# Autodesk Inventor assembly: underbrink_lite_asm_2
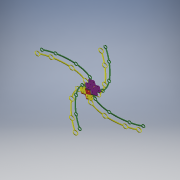
[picture p0: Inventor's stored thumbnail of the model, 180x180]
Saved by Autodesk Inventor 2019 (Build 230136000, 136)
## iProperties
Created: 2019-07-10
Part Number: underbrink_lite_asm_2
Document SubType Name: Assembly
Designer: Lino P
Mass: 5720.64 g
Surface Area: 2268.18 cm^2
Volume: 727.519 cm^3
Density: 7.86322 g/cm^3
Author: Lino P
## Documents named in this file (5)
- C:\Users\Lino P\Documents\000 - USFQ\TesisDev\ipt\underbrink_lite_asm_2.iam
- C:\Users\Lino P\Documents\000 - USFQ\TesisDev\ipt\underbrink_arm_lite_2.ipt
- C:\Users\Lino P\Documents\000 - USFQ\TesisDev\ipt\underbrink_base_lite.ipt
- C:\Users\Lino P\Documents\000 - USFQ\TesisDev\ipt\underbrink_arm_lite_2_bigDiam.ipt
- C:\Users\Lino P\Documents\000 - USFQ\TesisDev\ipt\underbrink_lite_asm_2\Design Accelerator\Shaft1.iam
## Components (26 placed, 4 different names)
1. underbrink_base_lite:1 — Mate:1, Mate:4, Mate:12
2. underbrink_base_lite:2 — Mate:13, Mate:14, Mate:20
3. underbrink_arm_lite_2:2 — Mate:1, Mate:4, Mate:12, Mate:16, Mate:17, Mate:18, Mate:23, Mate:26, Mate:27, Mate:28, Mate:29
4. underbrink_arm_lite_2:3
5. underbrink_arm_lite_2:4
6. underbrink_arm_lite_2:5
7. underbrink_arm_lite_2_bigDiam:1 — Mate:13, Mate:14, Mate:15, Mate:18, Mate:20, Mate:25
8. underbrink_arm_lite_2_bigDiam:2
9. underbrink_arm_lite_2_bigDiam:3
10. underbrink_arm_lite_2_bigDiam:4
11. Shaft:1 [sub-assembly] — Mate:15, Mate:16, Mate:17
12. Shaft:3 [sub-assembly] — Mate:23, Mate:27
13. Shaft:5 [sub-assembly] — Mate:25, Mate:26
14. Shaft:4 [sub-assembly] — Mate:28, Mate:29
15. Shaft:6 [sub-assembly]
16. Shaft:7 [sub-assembly]
17. Shaft:8 [sub-assembly]
18. Shaft:9 [sub-assembly]
19. Shaft:10 [sub-assembly]
20. Shaft:11 [sub-assembly]
21. Shaft:12 [sub-assembly]
22. Shaft:13 [sub-assembly]
23. Shaft:14 [sub-assembly]
24. Shaft:15 [sub-assembly]
25. Shaft:16 [sub-assembly]
26. Shaft:17 [sub-assembly]
## Component patterns: (4 elements, first: underbrink_arm_lite_2:2), (4 elements, first: underbrink_arm_lite_2_bigDiam:1), (4 elements, first: Shaft:1 + Shaft:3 + Shaft:5 + Shaft:4)
## Relationships (16: Mate 16)
- Mate:1: underbrink_base_lite:1 ↔ underbrink_arm_lite_2:2
- Mate:4: underbrink_base_lite:1 ↔ underbrink_arm_lite_2:2
- Mate:12: underbrink_base_lite:1 ↔ underbrink_arm_lite_2:2
- Mate:13: underbrink_base_lite:2 ↔ underbrink_arm_lite_2_bigDiam:1
- Mate:14: underbrink_base_lite:2 ↔ underbrink_arm_lite_2_bigDiam:1
- Mate:15: underbrink_arm_lite_2_bigDiam:1 ↔ Shaft:1
- Mate:16: underbrink_arm_lite_2:2 ↔ Shaft:1
- Mate:17: underbrink_arm_lite_2:2 ↔ Shaft:1
- Mate:18 (24 mm): underbrink_arm_lite_2:2 ↔ underbrink_arm_lite_2_bigDiam:1
- Mate:20: underbrink_base_lite:2 ↔ underbrink_arm_lite_2_bigDiam:1
- Mate:23: underbrink_arm_lite_2:2 ↔ Shaft:3
- Mate:25: underbrink_arm_lite_2_bigDiam:1 ↔ Shaft:5
- Mate:26: underbrink_arm_lite_2:2 ↔ Shaft:5
- Mate:27: underbrink_arm_lite_2:2 ↔ Shaft:3
- Mate:28: underbrink_arm_lite_2:2 ↔ Shaft:4
- Mate:29: underbrink_arm_lite_2:2 ↔ Shaft:4
